# Autodesk Inventor assembly: intento3
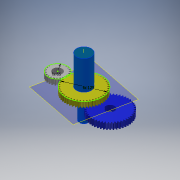
[picture p0: Inventor's stored thumbnail of the model, 180x180]
Saved by Autodesk Inventor 2019 (Build 230136000, 136)
## iProperties
Created: 2018-05-29
Part Number: intento3
Document SubType Name: Assembly
Designer: seba
Author: seba
## Documents named in this file (6)
- C:\Users\seba\Documents\Inventor\intento_engranes2\intento3.iam
- C:\Users\seba\Documents\Inventor\intento_engranes2\intento2\Design Accelerator\Spur Gears8.iam
- C:\Users\seba\Documents\Inventor\intento_engranes2\intento2\Design Accelerator\Spur Gears9.iam
- C:\Users\seba\Documents\Inventor\intento_engranes2\intento2\Design Accelerator\Spur Gears10.iam
- C:\Users\seba\Documents\Inventor\intento_engranes2\intento2\Design Accelerator\Spur Gear12.ipt
- C:\Users\seba\Documents\Inventor\intento_engranes2\eje_2_3.iam
## Components (5 placed, 3 different names)
1. Spur Gears:1 [sub-assembly] — Mate:1, Flush:1, Rotation:2
2. Spur Gears:2 [sub-assembly] — Flush:2, Mate:3, Mate:5, Flush:3, Rotation:1, Mate:10, Mate:11, Rotation:2
3. Spur Gears:3 [sub-assembly] — Mate:7, Mate:12, Mate:13, Rotation:3
4. Spur Gear1:1 — Mate:5, Mate:6, Rotation:1, Mate:9, Rotation:3
5. eje_2_3:1 [sub-assembly] — Mate:3, Mate:4
## Relationships (17: Mate 11, Flush 3, RelateRotation 3)
- Mate:1: Spur Gears:1
- Flush:1: Spur Gears:1
- Flush:2: Spur Gears:2
- Mate:3: Spur Gears:2 ↔ eje_2_3:1
- Mate:4: eje_2_3:1
- Mate:5: Spur Gears:2 ↔ Spur Gear1:1
- Mate:6: Spur Gear1:1
- Mate:7 (90 mm): Spur Gears:3
- Flush:3: Spur Gears:2
- Rotation:1 [RelateRotation] (1 ul): Spur Gears:2 ↔ Spur Gear1:1
- Mate:9: Spur Gear1:1
- Mate:10 (90 mm): Spur Gears:2
- Mate:11: Spur Gears:2
- Mate:12: Spur Gears:3
- Mate:13: Spur Gears:3
- Rotation:2 [RelateRotation] (2 ul): Spur Gears:1 ↔ Spur Gears:2
- Rotation:3 [RelateRotation] (2 ul): Spur Gears:3 ↔ Spur Gear1:1
